# Autodesk Inventor assembly: linear stepper
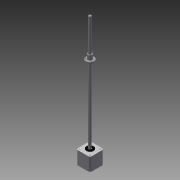
[picture p0: Inventor's stored thumbnail of the model, 180x180]
Saved by Autodesk Inventor 2015 (Build 190159000, 159)
## iProperties
Created: 2015-01-29
Part Number: linear stepper
Document SubType Name: Assembly
Designer: Joseph
Author: Joseph
## Documents named in this file (3)
- Z:\CloudStation\3d models\Kossel\linear stepper.iam
- Z:\CloudStation\3d models\Kossel\motor.ipt
- Z:\CloudStation\3d models\Kossel\lead carriage.ipt
## Components (2 placed, 2 different names)
1. motor:1 — Cylindrical:1
2. lead carriage:1 — Cylindrical:1
## Relationships (1: CylindricalJoint 1)
- Cylindrical:1: motor:1 ↔ lead carriage:1
